# Autodesk Inventor assembly: print008_Guss_mit_Einsatz
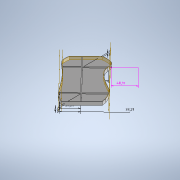
[picture p0: Inventor's stored thumbnail of the model, 180x180]
Saved by Autodesk Inventor 2020.3 (Build 243373000, 373)
## iProperties
Created: 2020-06-25
Part Number: print008_Guss_mit_Einsatz
Document SubType Name: Assembly
Designer: Mara
Mass: 14.6297 g
Surface Area: 295.485 cm^2
Volume: 14.6297 cm^3
Density: 1 g/cm^3
Author: Mara
## Documents named in this file (3)
- C:\Users\Mara\Masterarbeit_CAD\Guss_Löcher.iam
- C:\Users\Mara\Masterarbeit_CAD\Gussform.ipt
- C:\Users\Mara\Masterarbeit_CAD\Innenhalterung.ipt
## Components (2 placed, 2 different names)
1. Gussform:1
2. Innenhalterung:1 — Flush:1, Flush:2, Flush:3, Flush:4
## Relationships (4: Flush 4)
- Flush:1 (48.61 mm): Innenhalterung:1
- Flush:2 (47.67 mm): Innenhalterung:1
- Flush:3 (38.21 mm): Innenhalterung:1
- Flush:4 (32.91 mm): Innenhalterung:1
